# Autodesk Inventor assembly: 040400 DR-22-H4W(0.5)3
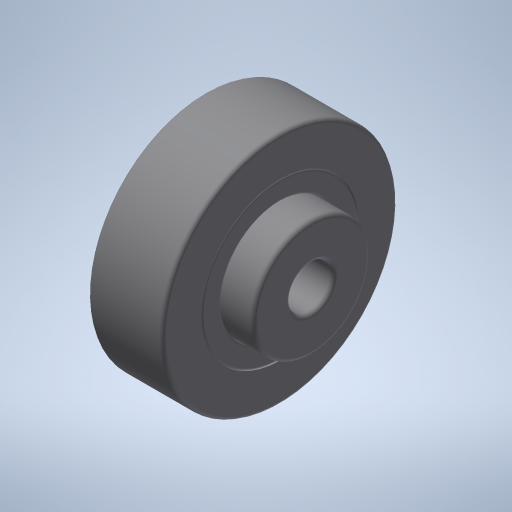
[picture p0: Inventor's stored thumbnail of the model, 512x512]
Saved by Autodesk Inventor 2024 (Build 280153000, 153)
## iProperties
Category: PARTsolutions
Created: 2023-06-17
Part Number: 040400 DR-22-H4W(0.5)3
Catalog Web Link: www.cadenas.de
Description: DR-H-
Document SubType Name: Assembly
Designer: psAdmin
Mass: 66400 g
Surface Area: 27.2924 cm^2
Volume: 2.61512 cm^3
Density: 25390.8 g/cm^3
PSOL_IDENT_0: {$CADENAS_DATA/23d-libs/tok_bearing/d_series_bearings/dr_h_asmtab.prj},189 {VTYP=3D},{STYP=ASSTAB},{
PSOL_IDENT_1: NB=040400 DR-22-H4W(0.5)3},{LINA=040400 DR-22-H4W(0.5)3},{NN=DR-H},{DATE=16.12.2020 00:38:04},{GEOMD
PSOL_IDENT_2: ATE=19.02.2013},{VERSION=},{LINEID=1750},{WBVAR=},{WBNUMERIC=}  {NB=040400 DR-22-H4W(0.5)3},{LINA=04
PSOL_IDENT_3: 0400 DR-22-H4W(0.5)3},{KT=DUMMY},{IDNR=},{CODE=040400},{PN=DR-22-H4W(0.5)3},{D=22},{SD=4.0},{W=7.0},
PSOL_IDENT_4: {W1=0.5},{W1X=0.500},{W2=3},{W2X=3.000},{LOAD=196 (20)},{TYPE=12},{QTY=1.000},{GW=8.3},{BD=3.78},{OP=
PSOL_IDENT_5: 40.2862},{N=5},{R=6.415},{GP=3.64},{PPATH=dr_h/dr_h_asmtpl.prj}
NB: 040400 DR-22-H4W(0.5)3
NN: DR-H
NBSYN: $CODE. $PN.
LINA: 040400 DR-22-H4W(0.5)3
CATALOG: TOK, Inc
CODE: 040400
PN: DR-22-H4W(0.5)3
D: 22
SD: 4
W: 7
W1: 0.5
W2: 3
LOAD: 196 (20)
TYPE: 12
QTY: 1.000
GW: 8.3
ARTICLENO: 040400 DR-22-H4W(0.5)3
BOMINFO: 040400 DR-22-H4W(0.5)3
CREATOR: CADENAS GmbH
Title: 040400 DR-22-H4W(0.5)3
Author: Cadenas PARTsolutions
## Documents named in this file (5)
- C:\Users\zegi\OneDrive - Kyushu University\KURT\2023キャチロボ\cad\000_parts_zegi\bearing\4\樹脂付きベアリング\040400 DR-22-H4W(0_5)3.iam
- C:\Users\zegi\OneDrive - Kyushu University\KURT\2023キャチロボ\cad\000_parts_zegi\bearing\4\樹脂付きベアリング\040400DR-22-H4W(0_5)3_ir.ipt
- C:\Users\zegi\OneDrive - Kyushu University\KURT\2023キャチロボ\cad\000_parts_zegi\bearing\4\樹脂付きベアリング\040400DR-22-H4W(0_5)3_or.ipt
- C:\Users\zegi\OneDrive - Kyushu University\KURT\2023キャチロボ\cad\000_parts_zegi\bearing\4\樹脂付きベアリング\040400DR-22-H4W(0_5)3_cage.ipt
- C:\Users\zegi\OneDrive - Kyushu University\KURT\2023キャチロボ\cad\000_parts_zegi\bearing\4\樹脂付きベアリング\040400DR-22-H4W(0_5)3_ball.ipt
## Components (8 placed, 4 different names)
1. 040400DR-22-H4W(0_5)3_ir:1 — IR_OR_XY@1 <-> OR_IR_XY@2, IR_OR_Z@1 <-> OR_IR_Z@2
2. 040400DR-22-H4W(0_5)3_or:1 — IR_OR_XY@1 <-> OR_IR_XY@2, IR_OR_Z@1 <-> OR_IR_Z@2, OR_IR_XY@2 <-> Cage_OR_XY@3, OR_IR_Z@2 <-> Cage_OR_Z@3, OR_ball_1_XY@2 <-> Ball_OR_XY@4, OR_ball_1_Z@2 <-> Ball_OR_Z@4, OR_ball_1_YZ@2 <-> Ball_OR_YZ@4, OR_ball_2_XY@2 <-> Ball_OR_XY@5, OR_ball_2_Z@2 <-> Ball_OR_Z@5, OR_ball_2_YZ@2 <-> Ball_OR_YZ@5, OR_ball_3_XY@2 <-> Ball_OR_XY@6, OR_ball_3_Z@2 <-> Ball_OR_Z@6, OR_ball_3_YZ@2 <-> Ball_OR_YZ@6, OR_ball_4_XY@2 <-> Ball_OR_XY@7, OR_ball_4_Z@2 <-> Ball_OR_Z@7, OR_ball_4_YZ@2 <-> Ball_OR_YZ@7, OR_ball_5_XY@2 <-> Ball_OR_XY@8, OR_ball_5_Z@2 <-> Ball_OR_Z@8, OR_ball_5_YZ@2 <-> Ball_OR_YZ@8, 対称度:1
3. 040400DR-22-H4W(0_5)3_cage:1 — OR_IR_XY@2 <-> Cage_OR_XY@3, OR_IR_Z@2 <-> Cage_OR_Z@3, 対称度:1
4. 040400DR-22-H4W(0_5)3_ball:1 — OR_ball_1_XY@2 <-> Ball_OR_XY@4, OR_ball_1_Z@2 <-> Ball_OR_Z@4, OR_ball_1_YZ@2 <-> Ball_OR_YZ@4
5. 040400DR-22-H4W(0_5)3_ball:2 — OR_ball_2_XY@2 <-> Ball_OR_XY@5, OR_ball_2_Z@2 <-> Ball_OR_Z@5, OR_ball_2_YZ@2 <-> Ball_OR_YZ@5
6. 040400DR-22-H4W(0_5)3_ball:3 — OR_ball_3_XY@2 <-> Ball_OR_XY@6, OR_ball_3_Z@2 <-> Ball_OR_Z@6, OR_ball_3_YZ@2 <-> Ball_OR_YZ@6
7. 040400DR-22-H4W(0_5)3_ball:4 — OR_ball_4_XY@2 <-> Ball_OR_XY@7, OR_ball_4_Z@2 <-> Ball_OR_Z@7, OR_ball_4_YZ@2 <-> Ball_OR_YZ@7
8. 040400DR-22-H4W(0_5)3_ball:5 — OR_ball_5_XY@2 <-> Ball_OR_XY@8, OR_ball_5_Z@2 <-> Ball_OR_Z@8, OR_ball_5_YZ@2 <-> Ball_OR_YZ@8
## Relationships (20: Mate 12, Angle 5, Flush 2, Symmetry 1)
- IR_OR_XY@1 <-> OR_IR_XY@2 [Flush]: 040400DR-22-H4W(0_5)3_ir:1 ↔ 040400DR-22-H4W(0_5)3_or:1
- IR_OR_Z@1 <-> OR_IR_Z@2 [Mate]: 040400DR-22-H4W(0_5)3_ir:1 ↔ 040400DR-22-H4W(0_5)3_or:1
- OR_IR_XY@2 <-> Cage_OR_XY@3 [Flush]: 040400DR-22-H4W(0_5)3_or:1 ↔ 040400DR-22-H4W(0_5)3_cage:1
- OR_IR_Z@2 <-> Cage_OR_Z@3 [Mate]: 040400DR-22-H4W(0_5)3_or:1 ↔ 040400DR-22-H4W(0_5)3_cage:1
- OR_ball_1_XY@2 <-> Ball_OR_XY@4 [Mate]: 040400DR-22-H4W(0_5)3_or:1 ↔ 040400DR-22-H4W(0_5)3_ball:1
- OR_ball_1_Z@2 <-> Ball_OR_Z@4 [Mate]: 040400DR-22-H4W(0_5)3_or:1 ↔ 040400DR-22-H4W(0_5)3_ball:1
- OR_ball_1_YZ@2 <-> Ball_OR_YZ@4 [Angle] (0 deg): 040400DR-22-H4W(0_5)3_or:1 ↔ 040400DR-22-H4W(0_5)3_ball:1
- OR_ball_2_XY@2 <-> Ball_OR_XY@5 [Mate]: 040400DR-22-H4W(0_5)3_or:1 ↔ 040400DR-22-H4W(0_5)3_ball:2
- OR_ball_2_Z@2 <-> Ball_OR_Z@5 [Mate]: 040400DR-22-H4W(0_5)3_or:1 ↔ 040400DR-22-H4W(0_5)3_ball:2
- OR_ball_2_YZ@2 <-> Ball_OR_YZ@5 [Angle] (0 deg): 040400DR-22-H4W(0_5)3_or:1 ↔ 040400DR-22-H4W(0_5)3_ball:2
- OR_ball_3_XY@2 <-> Ball_OR_XY@6 [Mate]: 040400DR-22-H4W(0_5)3_or:1 ↔ 040400DR-22-H4W(0_5)3_ball:3
- OR_ball_3_Z@2 <-> Ball_OR_Z@6 [Mate]: 040400DR-22-H4W(0_5)3_or:1 ↔ 040400DR-22-H4W(0_5)3_ball:3
- OR_ball_3_YZ@2 <-> Ball_OR_YZ@6 [Angle] (0 deg): 040400DR-22-H4W(0_5)3_or:1 ↔ 040400DR-22-H4W(0_5)3_ball:3
- OR_ball_4_XY@2 <-> Ball_OR_XY@7 [Mate]: 040400DR-22-H4W(0_5)3_or:1 ↔ 040400DR-22-H4W(0_5)3_ball:4
- OR_ball_4_Z@2 <-> Ball_OR_Z@7 [Mate]: 040400DR-22-H4W(0_5)3_or:1 ↔ 040400DR-22-H4W(0_5)3_ball:4
- OR_ball_4_YZ@2 <-> Ball_OR_YZ@7 [Angle] (0 deg): 040400DR-22-H4W(0_5)3_or:1 ↔ 040400DR-22-H4W(0_5)3_ball:4
- OR_ball_5_XY@2 <-> Ball_OR_XY@8 [Mate]: 040400DR-22-H4W(0_5)3_or:1 ↔ 040400DR-22-H4W(0_5)3_ball:5
- OR_ball_5_Z@2 <-> Ball_OR_Z@8 [Mate]: 040400DR-22-H4W(0_5)3_or:1 ↔ 040400DR-22-H4W(0_5)3_ball:5
- OR_ball_5_YZ@2 <-> Ball_OR_YZ@8 [Angle] (0 deg): 040400DR-22-H4W(0_5)3_or:1 ↔ 040400DR-22-H4W(0_5)3_ball:5
- 対称度:1 [Symmetry]: 040400DR-22-H4W(0_5)3_or:1 ↔ 040400DR-22-H4W(0_5)3_cage:1
